# Autodesk Inventor assembly: pullboxFiber
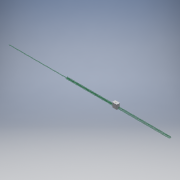
[picture p0: Inventor's stored thumbnail of the model, 180x180]
Saved by Autodesk Inventor 2017 (Build 210142000, 142)
## iProperties
Created: 2014-12-12
Part Number: pullboxFiber
Document SubType Name: Assembly
Designer: Dave
Author: Dave
## Documents named in this file (5)
- C:\Users\Kathryn Rosie\Google Drive\HERA\hera-cad\Node\pullboxFiber.iam
- C:\Users\Kathryn Rosie\Google Drive\HERA\hera-cad\Node\pullboxFiber.ipt
- C:\Users\Kathryn Rosie\Google Drive\HERA\hera-cad\Node\pipe_50mm_0.5m.ipt
- C:\Users\Kathryn Rosie\Google Drive\HERA\hera-cad\Node\pullboxFiberLid.ipt
- C:\Users\Kathryn Rosie\Google Drive\HERA\hera-cad\Node\pipe_50mm_Long.ipt
## Components (11 placed, 4 different names)
1. pullboxFiber:2 — Flush:1, Flush:2, Mate:1, Insert:6, Insert:7, Insert:8, Insert:9, Insert:10, Insert:11, Insert:12, Insert:13, Insert:14
2. pipe_50mm_0.5m:2 — Insert:6
3. pullboxFiberLid:1 — Flush:1, Flush:2, Mate:1
4. pipe_50mm_Long:1 — Insert:7
5. pipe_50mm_Long:2 — Insert:8
6. pipe_50mm_Long:3 — Insert:9
7. pipe_50mm_Long:4 — Insert:11
8. pipe_50mm_Long:5 — Insert:12
9. pipe_50mm_Long:6 — Insert:10
10. pipe_50mm_Long:7 — Insert:14
11. pipe_50mm_Long:8 — Insert:13
## Relationships (12: Insert 9, Flush 2, Mate 1)
- Flush:1: pullboxFiber:2 ↔ pullboxFiberLid:1
- Flush:2: pullboxFiber:2 ↔ pullboxFiberLid:1
- Mate:1 (5.08 mm): pullboxFiber:2 ↔ pullboxFiberLid:1
- Insert:6 (-254 mm): pullboxFiber:2 ↔ pipe_50mm_0.5m:2
- Insert:7 (-10000 mm): pullboxFiber:2 ↔ pipe_50mm_Long:1
- Insert:8 (-10000 mm): pullboxFiber:2 ↔ pipe_50mm_Long:2
- Insert:9 (-10000 mm): pullboxFiber:2 ↔ pipe_50mm_Long:3
- Insert:10 (-10000 mm): pullboxFiber:2 ↔ pipe_50mm_Long:6
- Insert:11 (-10000 mm): pullboxFiber:2 ↔ pipe_50mm_Long:4
- Insert:12 (-10000 mm): pullboxFiber:2 ↔ pipe_50mm_Long:5
- Insert:13: pullboxFiber:2 ↔ pipe_50mm_Long:8
- Insert:14: pullboxFiber:2 ↔ pipe_50mm_Long:7
